# Autodesk Inventor assembly: Butterfly Drive Module
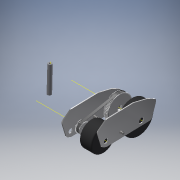
[picture p0: Inventor's stored thumbnail of the model, 180x180]
Saved by Autodesk Inventor 2019 (Build 230136000, 136)
## iProperties
Created: 2019-10-18
Part Number: Butterfly Drive Module
Document SubType Name: Assembly
Designer: admin
Author: admin
## Documents named in this file (9)
- C:\Users\Mark\Desktop\7738 Helion Engineering\7738-CAD-prep\Butterfly drive\Butterfly Drive Module.iam
- C:\Users\Mark\Desktop\7738 Helion Engineering\7738-CAD-prep\Butterfly drive\100mm Mecanum StandIn.ipt
- C:\Users\Mark\Desktop\7738 Helion Engineering\7738-CAD-prep\Butterfly drive\100mm Traction Wheel StandIn.ipt
- C:\Users\Mark\Desktop\7738 Helion Engineering\7738-CAD-prep\Butterfly drive\Butterfly Drive Module\Design Accelerator\Synchronous Belts Transmission3.iam
- C:\Users\Mark\Desktop\7738 Helion Engineering\7738-CAD-prep\Butterfly drive\F6800Z 10mm ID Flange.ipt
- C:\Users\Mark\Desktop\7738 Helion Engineering\7738-CAD-prep\Butterfly drive\Module Plate 1.ipt
- C:\Users\Mark\Desktop\7738 Helion Engineering\7738-CAD-prep\Butterfly drive\Stopper Axle.ipt
- C:\Users\Mark\Desktop\7738 Helion Engineering\7738-CAD-prep\Butterfly drive\Connector.ipt
- C:\Users\Mark\Desktop\7738 Helion Engineering\7738-CAD-prep\Butterfly drive\F6004.ipt
## Components (10 placed, 8 different names)
1. Connector:1 — Mate:34
2. 100mm Mecanum StandIn:1 — Flush:1, Mate:5, Mate:7, Angle:1
3. 100mm Traction Wheel StandIn:1 — Mate:4, Flush:1, Mate:6
4. Synchronous Belts Transmission:1 [sub-assembly] — Mate:5, Mate:6, Mate:7, Mate:15
5. F6800Z 10mm ID Flange:2 — Mate:15
6. Module Plate 1:1 — Mate:31, Mate:33, Insert:1
7. Module Plate 1:2 — Mate:32, Mate:33, Insert:2
8. Stopper Axle:1 — Mate:31, Mate:32
9. F6004:1 — Insert:1
10. F6004:2 — Insert:2
## Relationships (13: Mate 9, Insert 2, Flush 1, Angle 1)
- Mate:4: 100mm Traction Wheel StandIn:1
- Flush:1: 100mm Mecanum StandIn:1 ↔ 100mm Traction Wheel StandIn:1
- Mate:5: 100mm Mecanum StandIn:1 ↔ Synchronous Belts Transmission:1
- Mate:6: 100mm Traction Wheel StandIn:1 ↔ Synchronous Belts Transmission:1
- Mate:7 (2 mm): 100mm Mecanum StandIn:1 ↔ Synchronous Belts Transmission:1
- Angle:1 (90 deg): 100mm Mecanum StandIn:1
- Mate:15: Synchronous Belts Transmission:1 ↔ F6800Z 10mm ID Flange:2
- Mate:31: Module Plate 1:1 ↔ Stopper Axle:1
- Mate:32 (0.3 mm): Module Plate 1:2 ↔ Stopper Axle:1
- Mate:33 (105 mm): Module Plate 1:1 ↔ Module Plate 1:2
- Mate:34: Connector:1
- Insert:1: Module Plate 1:1 ↔ F6004:1
- Insert:2: Module Plate 1:2 ↔ F6004:2
